# Autodesk Inventor assembly: ProbeHead V2 TestAssembly
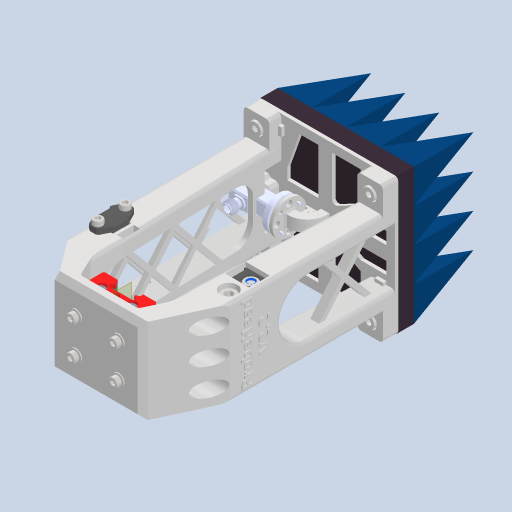
[picture p0: Inventor's stored thumbnail of the model, 512x512]
Saved by Autodesk Inventor 2023.2 (Build 272271000, 271)
## iProperties
Created: 2024-02-09
Part Number: ProbeHead V2 TestAssembly
Document SubType Name: Assembly
Designer: Nils Bade
Author: Nils Bade
## Documents named in this file (14)
- C:\Users\nilsb\Documents\Inventor\Projektarbeit-Bade\RatRig_modified\ProbeHead\ProbeHead V2 TestAssembly.iam
- C:\Users\nilsb\Documents\Inventor\Projektarbeit-Bade\RatRig_modified\MGN15 Linear-Rail-Block.ipt
- C:\Users\nilsb\Documents\Inventor\Projektarbeit-Bade\RatRig_Standards\face_belt_grabber v2.ipt
- C:\Users\nilsb\Documents\Inventor\Projektarbeit-Bade\Schrauben\Cap Head Screw M3x12 v2.ipt
- C:\Users\nilsb\Documents\Inventor\Projektarbeit-Bade\RatRig_Standards\Hex Nut - M3 v2.ipt
- C:\Users\nilsb\Documents\Inventor\Projektarbeit-Bade\Schrauben\Cap Head Screw M5x40 v2.ipt
- C:\Users\nilsb\Documents\Inventor\Projektarbeit-Bade\RatRig_Standards\Hex Locking Nut - M5 v2.ipt
- C:\Users\nilsb\Documents\Inventor\Projektarbeit-Bade\Schrauben\Cap Head Screw M4x12 - DIN912.ipt
- C:\Users\nilsb\Documents\Inventor\Projektarbeit-Bade\Schrauben\Washer Simple M3 - DIN6902.ipt
- C:\Users\nilsb\Documents\Inventor\Projektarbeit-Bade\RatRig_modified\ProbeHead\ProbeHead-Arms V2.ipt
- C:\Users\nilsb\Documents\Inventor\Projektarbeit-Bade\RatRig_modified\ProbeHead\Wire2Probe_Eravant_SWC-15VF-R1-V.ipt
- C:\Users\nilsb\Documents\Inventor\Projektarbeit-Bade\Enclosure\Absorber\Absorber - IHF-Mini.ipt
- C:\Users\nilsb\Documents\Inventor\Projektarbeit-Bade\RatRig_modified\core_xy_belt_grabber_Bade.ipt
- C:\Users\nilsb\Documents\Inventor\Projektarbeit-Bade\RatRig_modified\ProbeHead\ProbeAntennas\ProbeAntenna_V1.ipt
## Components (48 placed, 13 different names)
1. ProbeHead-Arms V2.2:1
2. core_xy_belt_grabber_Bade:2
3. core_xy_belt_grabber_Bade:1
4. MGN15 Linear-Rail-Block:1
5. face_belt_grabber v2:1 — Passend:16, Passend:17, Passend:18, Passend:19
6. face_belt_grabber v2:2 — Passend:12, Passend:13, Passend:14, Passend:15
7. Cap Head Screw M3x12 v2:1 — Passend:16, Passend:18, Passend:20
8. Cap Head Screw M3x12 v2:2 — Passend:17, Passend:19, Passend:21
9. Cap Head Screw M3x12 v2:3 — Passend:12, Passend:14, Passend:22
10. Cap Head Screw M3x12 v2:4 — Passend:13, Passend:15, Passend:23
11. Hex Nut - M3 v2:1 — Passend:20
12. Hex Nut - M3 v2:2 — Passend:23
13. Hex Nut - M3 v2:3 — Passend:22
14. Hex Nut - M3 v2:4 — Passend:21
15. Cap Head Screw M5x40 v2:1 — Passend:34
16. Cap Head Screw M5x40 v2:2
17. Hex Locking Nut - M5 v2:1
18. Hex Locking Nut - M5 v2:2 — Passend:34
19. Cap Head Screw M4x12 - DIN912:1
20. Cap Head Screw M4x12 - DIN912:2
21. Cap Head Screw M4x12 - DIN912:3
22. Cap Head Screw M4x12 - DIN912:4
23. Washer Simple M3 - DIN6902:1 — Passend:59
24. Washer Simple M3 - DIN6902:2 — Passend:56
25. Washer Simple M3 - DIN6902:3 — Passend:58
26. Washer Simple M3 - DIN6902:4 — Passend:57
27. Cap Head Screw M3x12 v2:5 — Passend:59
28. Cap Head Screw M3x12 v2:6 — Passend:58
29. Cap Head Screw M3x12 v2:7 — Passend:56
30. Cap Head Screw M3x12 v2:8 — Passend:57
31. ProbeAntenna V1:1
32. Wire2Probe_Eravant_SWC-15VF-R1-V:1
33. Absorber - IHF-Mini:1
34. Absorber - IHF-Mini:2
35. Absorber - IHF-Mini:3
36. Absorber - IHF-Mini:4
37. Absorber - IHF-Mini:5
38. Absorber - IHF-Mini:6
39. Absorber - IHF-Mini:7
40. Absorber - IHF-Mini:8
41. Absorber - IHF-Mini:9
42. Absorber - IHF-Mini:10
43. Absorber - IHF-Mini:11
44. Absorber - IHF-Mini:12
45. Absorber - IHF-Mini:13
46. Absorber - IHF-Mini:14
47. Absorber - IHF-Mini:15
48. Absorber - IHF-Mini:16
## Component patterns: (16 elements, first: Absorber - IHF-Mini:1)
## Relationships (78: Mate 64, Angle 8, Flush 6)
- [Mate]: ProbeHead-Arms V2.2:1 ↔ MGN15 Linear-Rail-Block:1
- [Mate]: ProbeHead-Arms V2.2:1 ↔ MGN15 Linear-Rail-Block:1
- [Mate]: ProbeHead-Arms V2.2:1 ↔ MGN15 Linear-Rail-Block:1
- [Mate]: ProbeHead-Arms V2.2:1 ↔ core_xy_belt_grabber_Bade:1
- [Angle] (0 deg): ProbeHead-Arms V2.2:1 ↔ core_xy_belt_grabber_Bade:2
- [Mate]: ProbeHead-Arms V2.2:1 ↔ core_xy_belt_grabber_Bade:2
- [Flush] (2 mm): ProbeHead-Arms V2.2:1 ↔ core_xy_belt_grabber_Bade:2
- [Flush] (2 mm): ProbeHead-Arms V2.2:1 ↔ core_xy_belt_grabber_Bade:1
- [Mate]: ProbeHead-Arms V2.2:1 ↔ face_belt_grabber v2:2
- [Mate]: ProbeHead-Arms V2.2:1 ↔ face_belt_grabber v2:2
- [Mate]: ProbeHead-Arms V2.2:1 ↔ face_belt_grabber v2:1
- [Mate]: ProbeHead-Arms V2.2:1 ↔ face_belt_grabber v2:1
- Passend:12 [Mate]: face_belt_grabber v2:2 ↔ Cap Head Screw M3x12 v2:3
- Passend:13 [Mate]: face_belt_grabber v2:2 ↔ Cap Head Screw M3x12 v2:4
- Passend:14 [Mate]: face_belt_grabber v2:2 ↔ Cap Head Screw M3x12 v2:3
- Passend:15 [Mate]: face_belt_grabber v2:2 ↔ Cap Head Screw M3x12 v2:4
- Passend:16 [Mate]: face_belt_grabber v2:1 ↔ Cap Head Screw M3x12 v2:1
- Passend:17 [Mate]: face_belt_grabber v2:1 ↔ Cap Head Screw M3x12 v2:2
- Passend:18 [Mate]: face_belt_grabber v2:1 ↔ Cap Head Screw M3x12 v2:1
- Passend:19 [Mate]: face_belt_grabber v2:1 ↔ Cap Head Screw M3x12 v2:2
- Passend:20 [Mate]: Cap Head Screw M3x12 v2:1 ↔ Hex Nut - M3 v2:1
- Passend:21 [Mate]: Cap Head Screw M3x12 v2:2 ↔ Hex Nut - M3 v2:4
- Passend:22 [Mate]: Cap Head Screw M3x12 v2:3 ↔ Hex Nut - M3 v2:3
- Passend:23 [Mate]: Cap Head Screw M3x12 v2:4 ↔ Hex Nut - M3 v2:2
- [Angle] (0 deg): ProbeHead-Arms V2.2:1 ↔ Hex Nut - M3 v2:1
- [Angle] (0 deg): ProbeHead-Arms V2.2:1 ↔ Hex Nut - M3 v2:3
- [Mate]: ProbeHead-Arms V2.2:1 ↔ Hex Nut - M3 v2:3
- [Mate]: ProbeHead-Arms V2.2:1 ↔ Hex Nut - M3 v2:2
- [Mate]: ProbeHead-Arms V2.2:1 ↔ Hex Nut - M3 v2:1
- [Mate]: ProbeHead-Arms V2.2:1 ↔ Hex Nut - M3 v2:4
- [Mate]: ProbeHead-Arms V2.2:1 ↔ Cap Head Screw M5x40 v2:2
- [Mate]: ProbeHead-Arms V2.2:1 ↔ Cap Head Screw M5x40 v2:1
- [Mate]: ProbeHead-Arms V2.2:1 ↔ Cap Head Screw M5x40 v2:1
- [Mate]: ProbeHead-Arms V2.2:1 ↔ Cap Head Screw M5x40 v2:2
- [Mate]: core_xy_belt_grabber_Bade:1 ↔ Hex Locking Nut - M5 v2:1
- [Mate]: core_xy_belt_grabber_Bade:1 ↔ Hex Locking Nut - M5 v2:1
- Passend:34 [Mate]: Cap Head Screw M5x40 v2:1 ↔ Hex Locking Nut - M5 v2:2
- [Angle] (0 deg): core_xy_belt_grabber_Bade:2 ↔ Hex Locking Nut - M5 v2:2
- [Mate]: core_xy_belt_grabber_Bade:2 ↔ Hex Locking Nut - M5 v2:2
- [Angle] (0 deg): core_xy_belt_grabber_Bade:1 ↔ Hex Locking Nut - M5 v2:1
- [Mate]: ProbeHead-Arms V2.2:1 ↔ Cap Head Screw M4x12 - DIN912:1
- [Mate]: ProbeHead-Arms V2.2:1 ↔ Cap Head Screw M4x12 - DIN912:2
- [Mate]: ProbeHead-Arms V2.2:1 ↔ Cap Head Screw M4x12 - DIN912:4
- [Mate]: ProbeHead-Arms V2.2:1 ↔ Cap Head Screw M4x12 - DIN912:3
- [Mate]: ProbeHead-Arms V2.2:1 ↔ Cap Head Screw M4x12 - DIN912:1
- [Mate]: ProbeHead-Arms V2.2:1 ↔ Cap Head Screw M4x12 - DIN912:2
- [Mate]: ProbeHead-Arms V2.2:1 ↔ Cap Head Screw M4x12 - DIN912:4
- [Mate]: ProbeHead-Arms V2.2:1 ↔ Cap Head Screw M4x12 - DIN912:3
- [Mate]: ProbeHead-Arms V2.2:1 ↔ Washer Simple M3 - DIN6902:1
- [Mate]: ProbeHead-Arms V2.2:1 ↔ Washer Simple M3 - DIN6902:2
- [Mate]: ProbeHead-Arms V2.2:1 ↔ Washer Simple M3 - DIN6902:3
- [Mate]: ProbeHead-Arms V2.2:1 ↔ Washer Simple M3 - DIN6902:4
- [Mate]: ProbeHead-Arms V2.2:1 ↔ Washer Simple M3 - DIN6902:4
- [Mate]: ProbeHead-Arms V2.2:1 ↔ Washer Simple M3 - DIN6902:2
- [Mate]: ProbeHead-Arms V2.2:1 ↔ Washer Simple M3 - DIN6902:1
- [Mate]: ProbeHead-Arms V2.2:1 ↔ Washer Simple M3 - DIN6902:3
- [Mate]: ProbeHead-Arms V2.2:1 ↔ Cap Head Screw M3x12 v2:5
- [Mate]: ProbeHead-Arms V2.2:1 ↔ Cap Head Screw M3x12 v2:6
- [Mate]: ProbeHead-Arms V2.2:1 ↔ Cap Head Screw M3x12 v2:7
- [Mate]: ProbeHead-Arms V2.2:1 ↔ Cap Head Screw M3x12 v2:8
- Passend:56 [Mate]: Washer Simple M3 - DIN6902:2 ↔ Cap Head Screw M3x12 v2:7
- Passend:57 [Mate]: Washer Simple M3 - DIN6902:4 ↔ Cap Head Screw M3x12 v2:8
- Passend:58 [Mate]: Washer Simple M3 - DIN6902:3 ↔ Cap Head Screw M3x12 v2:6
- Passend:59 [Mate]: Washer Simple M3 - DIN6902:1 ↔ Cap Head Screw M3x12 v2:5
- [Mate]: ProbeHead-Arms V2.2:1 ↔ Cap Head Screw M3x12 v2:4
- [Mate]: ProbeHead-Arms V2.2:1 ↔ Cap Head Screw M3x12 v2:2
- [Angle] (0 deg): ProbeHead-Arms V2.2:1 ↔ Hex Nut - M3 v2:2
- [Angle] (0 deg): ProbeHead-Arms V2.2:1 ↔ Hex Nut - M3 v2:4
- [Mate]: Cap Head Screw M4x12 - DIN912:4 ↔ ProbeAntenna V1:1
- [Mate]: Cap Head Screw M4x12 - DIN912:1 ↔ ProbeAntenna V1:1
- [Flush]: ProbeAntenna V1:1 ↔ Wire2Probe_Eravant_SWC-15VF-R1-V:1
- [Flush]: ProbeAntenna V1:1 ↔ Wire2Probe_Eravant_SWC-15VF-R1-V:1
- [Mate]: ProbeAntenna V1:1 ↔ Wire2Probe_Eravant_SWC-15VF-R1-V:1
- [Mate]: ProbeHead-Arms V2.2:1 ↔ ProbeAntenna V1:1
- [Mate]: ProbeAntenna V1:1 ↔ Absorber - IHF-Mini:1
- [Flush]: ProbeAntenna V1:1 ↔ Absorber - IHF-Mini:1
- [Flush] (0.85 mm): ProbeAntenna V1:1 ↔ Absorber - IHF-Mini:1
- [Angle] (180 deg): ProbeHead-Arms V2.2:1 ↔ core_xy_belt_grabber_Bade:1
